# Autodesk Inventor assembly: CARCASA_ESTRUCTURA_Y_CHAPAS
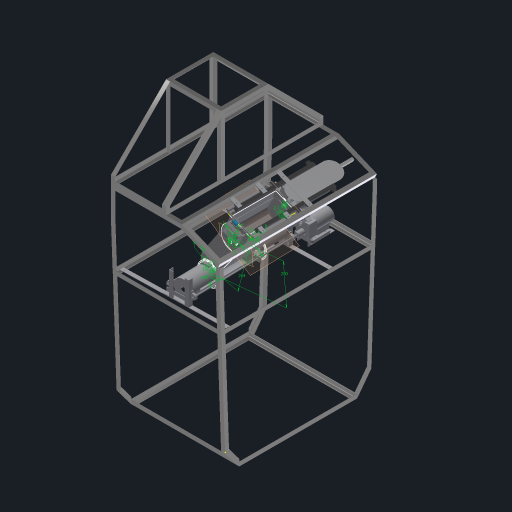
[picture p0: Inventor's stored thumbnail of the model, 512x512]
Saved by Autodesk Inventor 2024.3 (Build 283343000, 343)
## iProperties
Created: 2024-05-18
Part Number: CARCASA_ESTRUCTURA_Y_CHAPAS
Material: Generic
Document SubType Name: Assembly
Designer: Niler
Author: Niler
## Documents named in this file (7)
- C:\Users\Niler\OneDrive\Escritorio\RECICLADOR\RECICLADOR_MODELO_3D\VERSION_3_COMPLETA\CARCASA_ESTRUCTURA_Y_CHAPAS_1.iam
- C:\Users\Niler\OneDrive\Escritorio\RECICLADOR\RECICLADOR_MODELO_3D\VERSION_3_COMPLETA\ESTRUCTURA\ESTRUCTURA_COMPLETA.iam
- C:\Users\Niler\OneDrive\Escritorio\RECICLADOR\RECICLADOR_MODELO_3D\MECANISMO DE COMPACTADO\ENSAMBLE MECANISMO DE INGRESO.iam
- C:\Users\Niler\OneDrive\Escritorio\RECICLADOR\RECICLADOR_MODELO_3D\MECANISMO DE COMPACTADO\MECANISMO DE COMPACTADO.iam
- C:\Users\Niler\OneDrive\Escritorio\RECICLADOR\RECICLADOR_MODELO_3D\MECANISMO DE COMPACTADO\SOPORTE INERCIAL DE LA CAJA SEPARADORA.ipt
- C:\Users\Niler\OneDrive\Escritorio\RECICLADOR\RECICLADOR_MODELO_3D\VERSION_3_COMPLETA\CANALETA_GUIA.ipt
- C:\Users\Niler\OneDrive\Escritorio\RECICLADOR\RECICLADOR_MODELO_3D\VERSION_3_COMPLETA\SEGURO_CANALETA.ipt
## Components (7 placed, 6 different names)
1. ESTRUCTURA_COMPLETA:1 [sub-assembly] — Mate:13, Mate:14, Mate:15, Mate:23
2. ENSAMBLE MECANISMO DE INGRESO:1 [sub-assembly] — Mate:14, Mate:15
3. MECANISMO DE COMPACTADO:1 [sub-assembly] — Mate:23, Mate:24
4. SOPORTE INERCIAL DE LA CAJA SEPARADORA:1 — Mate:13
5. CANALETA_GUIA:1 — Mate:17, Mate:18, Mate:19, Mate:20, Mate:21, Mate:22
6. SEGURO_CANALETA:1 — Mate:20, Mate:21, Mate:22, Mate:24
7. SEGURO_CANALETA:2 — Mate:17, Mate:18, Mate:19
## Relationships (11: Mate 11)
- Mate:13: ESTRUCTURA_COMPLETA:1 ↔ SOPORTE INERCIAL DE LA CAJA SEPARADORA:1
- Mate:14: ESTRUCTURA_COMPLETA:1 ↔ ENSAMBLE MECANISMO DE INGRESO:1
- Mate:15: ESTRUCTURA_COMPLETA:1 ↔ ENSAMBLE MECANISMO DE INGRESO:1
- Mate:17: CANALETA_GUIA:1 ↔ SEGURO_CANALETA:2
- Mate:18: CANALETA_GUIA:1 ↔ SEGURO_CANALETA:2
- Mate:19: CANALETA_GUIA:1 ↔ SEGURO_CANALETA:2
- Mate:20: CANALETA_GUIA:1 ↔ SEGURO_CANALETA:1
- Mate:21: CANALETA_GUIA:1 ↔ SEGURO_CANALETA:1
- Mate:22: CANALETA_GUIA:1 ↔ SEGURO_CANALETA:1
- Mate:23: ESTRUCTURA_COMPLETA:1 ↔ MECANISMO DE COMPACTADO:1
- Mate:24: MECANISMO DE COMPACTADO:1 ↔ SEGURO_CANALETA:1
